# Autodesk Inventor assembly: F-wing
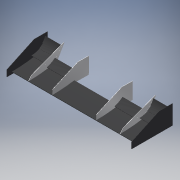
[picture p0: Inventor's stored thumbnail of the model, 180x180]
Saved by Autodesk Inventor 2018.1 (Build 221171000, 171)
## iProperties
Created: 2017-10-18
Part Number: F-wing
Material: 一般
Document SubType Name: Assembly
Designer: kuwano
Mass: 4818.18 g
Surface Area: 15581.9 cm^2
Volume: 2926.88 cm^3
Density: 1.64618 g/cm^3
Author: kuwano
## Documents named in this file (8)
- D:\ku_sk\ドキュメント\Inventor\KS-15_Aero_CAD\type4\F-wing\F-wing.iam
- D:\ku_sk\ドキュメント\Inventor\KS-15_Aero_CAD\type4\F-wing\parts\side.ipt
- D:\ku_sk\ドキュメント\Inventor\KS-15_Aero_CAD\type4\F-wing\parts\element_1.ipt
- D:\ku_sk\ドキュメント\Inventor\KS-15_Aero_CAD\type4\F-wing\parts\element_2.ipt
- D:\ku_sk\ドキュメント\Inventor\KS-15_Aero_CAD\type4\F-wing\parts\stay_middle.ipt
- D:\ku_sk\ドキュメント\Inventor\KS-15_Aero_CAD\type4\F-wing\parts\base.ipt
- D:\ku_sk\ドキュメント\Inventor\KS-15_Aero_CAD\type4\F-wing\parts\element_4.ipt
- D:\ku_sk\ドキュメント\Inventor\KS-15_Aero_CAD\type4\F-wing\parts\stay.ipt
## Components (15 placed, 7 different names)
1. side:2 — メイト:10, フラッシュ:14, フラッシュ:15, メイト:24, メイト:25, メイト:38, 角度:2
2. side:4 — メイト:7, フラッシュ:14, フラッシュ:15, メイト:22, メイト:23, メイト:39, メイト:43
3. element_1:1 — メイト:10, メイト:17, フラッシュ:12, メイト:27
4. element_1:2 — メイト:7, メイト:17, フラッシュ:12, メイト:26
5. element_2:1 — フラッシュ:11, メイト:15, メイト:25
6. element_2:2 — フラッシュ:10, メイト:16, メイト:24
7. element_2:3 — フラッシュ:11, メイト:15, メイト:23
8. element_2:4 — フラッシュ:10, メイト:16, メイト:22
9. element_4:1 — メイト:30, メイト:42, フラッシュ:41
10. element_4:2 — メイト:32, メイト:42, フラッシュ:41
11. stay_middle:1 — フラッシュ:16, フラッシュ:17, メイト:27, メイト:32
12. stay_middle:2 — フラッシュ:16, フラッシュ:17, メイト:26, メイト:30, メイト:44, メイト:45, 角度:3
13. base:1 — フラッシュ:18, メイト:38, メイト:39, メイト:40, メイト:41, メイト:43, メイト:44, メイト:45, 角度:1
14. stay:1 — フラッシュ:39, フラッシュ:40
15. stay:2 — フラッシュ:39, フラッシュ:40, メイト:40, メイト:41
## Relationships (35: Mate 21, Flush 11, Angle 3)
- メイト:7 [Mate]: side:4 ↔ element_1:2
- メイト:10 [Mate]: side:2 ↔ element_1:1
- フラッシュ:10 [Flush]: element_2:2 ↔ element_2:4
- フラッシュ:11 [Flush]: element_2:1 ↔ element_2:3
- メイト:15 [Mate]: element_2:1 ↔ element_2:3
- メイト:16 [Mate]: element_2:2 ↔ element_2:4
- メイト:17 [Mate]: element_1:1 ↔ element_1:2
- フラッシュ:12 [Flush]: element_1:1 ↔ element_1:2
- フラッシュ:14 [Flush]: side:2 ↔ side:4
- フラッシュ:15 [Flush]: side:2 ↔ side:4
- フラッシュ:16 [Flush]: stay_middle:1 ↔ stay_middle:2
- フラッシュ:17 [Flush]: stay_middle:1 ↔ stay_middle:2
- メイト:22 [Mate]: side:4 ↔ element_2:4
- メイト:23 [Mate]: side:4 ↔ element_2:3
- メイト:24 [Mate]: side:2 ↔ element_2:2
- メイト:25 [Mate]: side:2 ↔ element_2:1
- メイト:26 [Mate]: element_1:2 ↔ stay_middle:2
- メイト:27 [Mate]: element_1:1 ↔ stay_middle:1
- フラッシュ:18 [Flush]: base:1
- メイト:30 [Mate]: element_4:1 ↔ stay_middle:2
- メイト:32 [Mate]: element_4:2 ↔ stay_middle:1
- フラッシュ:39 [Flush]: stay:1 ↔ stay:2
- フラッシュ:40 [Flush]: stay:1 ↔ stay:2
- メイト:38 [Mate]: side:2 ↔ base:1
- メイト:39 [Mate]: side:4 ↔ base:1
- メイト:40 [Mate]: base:1 ↔ stay:2
- メイト:41 [Mate]: base:1 ↔ stay:2
- メイト:42 [Mate]: element_4:1 ↔ element_4:2
- フラッシュ:41 [Flush]: element_4:1 ↔ element_4:2
- メイト:43 [Mate] (-20 mm): side:4 ↔ base:1
- メイト:44 [Mate]: stay_middle:2 ↔ base:1
- メイト:45 [Mate]: stay_middle:2 ↔ base:1
- 角度:1 [Angle] (0 deg): base:1
- 角度:2 [Angle] (0 deg): side:2
- 角度:3 [Angle] (0 deg): stay_middle:2
